# Autodesk Inventor assembly: servo grab
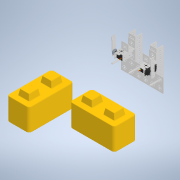
[picture p0: Inventor's stored thumbnail of the model, 180x180]
Saved by Autodesk Inventor 2020 (Build 240168000, 168)
## iProperties
Created: 2019-09-14
Part Number: servo grab
Document SubType Name: Assembly
Designer: tbloo
Author: tbloo
## Documents named in this file (10)
- D:\Documents\GitHub\AO_Robotics\CAD\Projects\Timothy Bloot\servo grab.iam
- D:\Documents\GitHub\AO_Robotics\CAD\Parts Kits\FTC Tetrix KOP Organized (7-24-19)\Stand-off posts\Tetrix_39103.ipt
- D:\Documents\GitHub\AO_Robotics\CAD\Parts Kits\FTC Tetrix KOP Organized (7-24-19)\Frame Hardware\Tetrix_39073.ipt
- D:\Documents\GitHub\AO_Robotics\CAD\Skystone Field\1x2 Block v2.ipt
- D:\Documents\GitHub\AO_Robotics\CAD\Parts Kits\FTC Tetrix KOP Organized (7-24-19)\Servo\Tetrix_39060.ipt
- D:\Documents\GitHub\AO_Robotics\CAD\Parts Kits\FTC Tetrix KOP Organized (7-24-19)\Servo\Tetrix_39197_Servo.ipt
- D:\Documents\GitHub\AO_Robotics\CAD\Parts Kits\FTC Tetrix KOP Organized (7-24-19)\Frame Hardware\Tetrix_39065.ipt
- D:\Documents\GitHub\AO_Robotics\CAD\Parts Kits\FTC Tetrix KOP Organized (7-24-19)\Frame Hardware\Tetrix_39067.ipt
- D:\Documents\GitHub\AO_Robotics\CAD\Projects\Timothy Bloot\Tetrix_3907-5.ipt
- D:\Documents\GitHub\AO_Robotics\CAD\Parts Kits\FTC Tetrix KOP Organized (7-24-19)\Servo\Tetrix_39197_Metal_Horn.ipt
## Components (18 placed, 9 different names)
1. Tetrix_39103:1 — Rigid:8
2. Tetrix_39103:2 — Rigid:2
3. Tetrix_39103:3 — Rigid:1
4. Tetrix_39073:1 — Rigid:1, Rigid:2, Rigid:5, Rigid:8, Rigid:9
5. 1x2 Block v2:1
6. Tetrix_39060:1 — Rigid:6, Rigid:7
7. Tetrix_39067:1 — Rigid:5, Mate:2, Rigid:13
8. Tetrix_39065:2 — Rigid:6, Mate:2, Rigid:13
9. Tetrix_39197_Servo:1 — Rigid:7, Rotational:1
10. 1x2 Block v2:2
11. Tetrix_39067:2 — Rigid:12, Rigid:9
12. Tetrix_39065:3 — Rigid:12, Rigid:10
13. Tetrix_39060:2 — Rigid:10, Rigid:11
14. Tetrix_39197_Servo:2 — Rigid:11, Rotational:2
15. Tetrix_39197_Metal_Horn:1 — Rotational:1, Rigid:14
16. Tetrix_39197_Metal_Horn:2 — Rotational:2, Rigid:15
17. Tetrix_3907-5:1 — Rigid:14, Cylindrical:1
18. Tetrix_3907-5:2 — Rigid:15, Cylindrical:1
## Relationships (18: WeldJoint 13, Mate 2, RevoluteJoint 2, CylindricalJoint 1)
- Rigid:1 [WeldJoint]: Tetrix_39103:3 ↔ Tetrix_39073:1
- Rigid:2 [WeldJoint]: Tetrix_39103:2 ↔ Tetrix_39073:1
- Rigid:5 [WeldJoint]: Tetrix_39073:1 ↔ Tetrix_39067:1
- Rigid:6 [WeldJoint]: Tetrix_39060:1 ↔ Tetrix_39065:2
- Mate:2: Tetrix_39067:1 ↔ Tetrix_39065:2
- Rigid:13 [WeldJoint]: Tetrix_39067:1 ↔ Tetrix_39065:2
- Rigid:7 [WeldJoint]: Tetrix_39060:1 ↔ Tetrix_39197_Servo:1
- Rigid:8 [WeldJoint]: Tetrix_39103:1 ↔ Tetrix_39073:1
- [Mate]: Tetrix_39067:2 ↔ Tetrix_39065:3
- Rigid:12 [WeldJoint]: Tetrix_39067:2 ↔ Tetrix_39065:3
- Rigid:9 [WeldJoint]: Tetrix_39073:1 ↔ Tetrix_39067:2
- Rigid:10 [WeldJoint]: Tetrix_39065:3 ↔ Tetrix_39060:2
- Rigid:11 [WeldJoint]: Tetrix_39060:2 ↔ Tetrix_39197_Servo:2
- Rotational:1 [RevoluteJoint]: Tetrix_39197_Servo:1 ↔ Tetrix_39197_Metal_Horn:1
- Rotational:2 [RevoluteJoint]: Tetrix_39197_Servo:2 ↔ Tetrix_39197_Metal_Horn:2
- Rigid:14 [WeldJoint]: Tetrix_39197_Metal_Horn:1 ↔ Tetrix_3907-5:1
- Rigid:15 [WeldJoint]: Tetrix_39197_Metal_Horn:2 ↔ Tetrix_3907-5:2
- Cylindrical:1: Tetrix_3907-5:1 ↔ Tetrix_3907-5:2
## Named parameters: d20_d15 = 0 mm, d21_d16 = 0 mm, d22_d17 = 0 deg
